# Autodesk Inventor assembly: Digester2
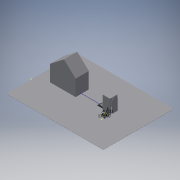
[picture p0: Inventor's stored thumbnail of the model, 180x180]
Saved by Autodesk Inventor 2019 (Build 230136000, 136)
## iProperties
Created: 2019-11-06
Part Number: Digester2
Document SubType Name: Assembly
Designer: Administrator
Author: Administrator
## Documents named in this file (10)
- H:\CAD30\Digester2.iam
- H:\CAD30\dome.ipt
- H:\CAD30\mock ground.ipt
- H:\CAD30\pOOPOODOOR.ipt
- C:\Users\manwer\Downloads\Base (1).ipt
- C:\Users\manwer\Downloads\Lid (1).ipt
- H:\CAD30\pipenew.ipt
- H:\CAD30\fonl.ipt
- H:\CAD30\tbe.ipt
- H:\CAD30\another tube.ipt
## Components (9 placed, 9 different names)
1. dome:1
2. mock ground:1 — Flush:1, Mate:4, Mate:5, Flush:2
3. pOOPOODOOR:1 — Flush:1
4. Base (1):1 — Mate:2, Mate:3
5. Lid (1):1 — Mate:2, Mate:3
6. pipenew:1
7. fonl:1 — Mate:4, Mate:5
8. tbe:1 — Flush:2
9. another tube:1
## Relationships (6: Mate 4, Flush 2)
- Flush:1: mock ground:1 ↔ pOOPOODOOR:1
- Mate:2: Base (1):1 ↔ Lid (1):1
- Mate:3: Base (1):1 ↔ Lid (1):1
- Mate:4: mock ground:1 ↔ fonl:1
- Mate:5: mock ground:1 ↔ fonl:1
- Flush:2: mock ground:1 ↔ tbe:1
